# Autodesk Inventor assembly: am14u3LongWithRevForkLift
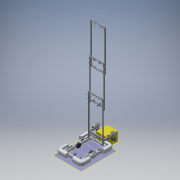
[picture p0: Inventor's stored thumbnail of the model, 180x180]
Saved by Autodesk Inventor 2019.3 (Build 233278000, 278)
## iProperties
Created: 2018-01-15
Part Number: am14u3LongWithRevForkLift
Document SubType Name: Assembly
Designer: steele
Author: steele
## Documents named in this file (5)
- C:\git\CAD-Development\robSteele\2018-FRC\am14u3LongWithRevForkLift.iam
- C:\git\CAD-Development\robSteele\2018-FRC\AMbaseLongWithBumper\Long with Bumper\DB_DriveBaseLong_AM14U3_Bumpers and Battery Tray.iam
- C:\git\CAD-Development\robSteele\2018-FRC\RevRobotics\REV-25-1238-1239.iam
- C:\git\CAD-Development\robSteele\2018-FRC\Field Elements\Cube-GE-18124.ipt
- C:\git\CAD-Development\robSteele\2018-FRC\Gripper\gripperAssembly.iam
## Components (4 placed, 4 different names)
1. DB_DriveBaseLong_AM14U3_Bumpers and Battery Tray:1 [sub-assembly] — Mate:1, Flush:1, Mate:2, Flush:2, Mate:3, Mate:4, Mate:5, Mate:7
2. REV-25-1238-1239:1 [sub-assembly] — Mate:1, Flush:1, Mate:2, Mate:8
3. Cube-GE-18124:1 — Mate:3, Mate:4, Mate:5
4. gripperAssembly:1 [sub-assembly] — Mate:6, Mate:7, Mate:8
## Relationships (10: Mate 8, Flush 2)
- Mate:1: DB_DriveBaseLong_AM14U3_Bumpers and Battery Tray:1 ↔ REV-25-1238-1239:1
- Flush:1: DB_DriveBaseLong_AM14U3_Bumpers and Battery Tray:1 ↔ REV-25-1238-1239:1
- Mate:2: DB_DriveBaseLong_AM14U3_Bumpers and Battery Tray:1 ↔ REV-25-1238-1239:1
- Flush:2 (50.8 mm): DB_DriveBaseLong_AM14U3_Bumpers and Battery Tray:1
- Mate:3: DB_DriveBaseLong_AM14U3_Bumpers and Battery Tray:1 ↔ Cube-GE-18124:1
- Mate:4: DB_DriveBaseLong_AM14U3_Bumpers and Battery Tray:1 ↔ Cube-GE-18124:1
- Mate:5: DB_DriveBaseLong_AM14U3_Bumpers and Battery Tray:1 ↔ Cube-GE-18124:1
- Mate:6 (-279.4 mm): gripperAssembly:1
- Mate:7: DB_DriveBaseLong_AM14U3_Bumpers and Battery Tray:1 ↔ gripperAssembly:1
- Mate:8: REV-25-1238-1239:1 ↔ gripperAssembly:1
